# Autodesk Inventor assembly: RMTestMachine
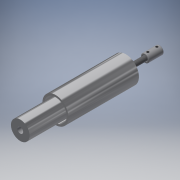
[picture p0: Inventor's stored thumbnail of the model, 180x180]
Saved by Autodesk Inventor 2019 (Build 230136000, 136)
## iProperties
Created: 2019-05-15
Part Number: RMTestMachine
Document SubType Name: Assembly
Designer: Iván
Author: Iván
## Documents named in this file (5)
- C:\Users\Iván\Documents\Github\RMTestMachine\3DModel\RMTestMachine.iam
- C:\Users\Iván\Documents\Github\RMTestMachine\3DModel\AcopleMotor.ipt
- C:\Users\Iván\Documents\Github\RMTestMachine\3DModel\BarraRoscadaT8.ipt
- C:\Users\Iván\Documents\Github\RMTestMachine\3DModel\BarraSolidaMotor.ipt
- C:\Users\Iván\Documents\Github\RMTestMachine\3DModel\TuboSoporte.ipt
## Components (4 placed, 4 different names)
1. AcopleMotor:1 — Insert:1
2. BarraRoscadaT8:1 — Insert:1, Rotation/Translation:1
3. BarraSolidaMotor:1 — Rotation/Translation:1, Insert:2
4. TuboSoporte:1 — Insert:2
## Relationships (3: Insert 2, RelateRotateTranslate 1)
- Insert:1 (12.7 mm): AcopleMotor:1 ↔ BarraRoscadaT8:1
- Rotation/Translation:1 [RelateRotateTranslate] (150 mm): BarraRoscadaT8:1 ↔ BarraSolidaMotor:1
- Insert:2 (-180 mm): BarraSolidaMotor:1 ↔ TuboSoporte:1
